# Autodesk Inventor assembly: Carriage_Assembly
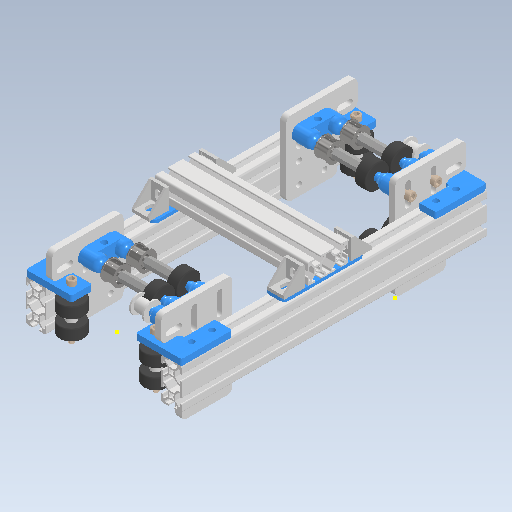
[picture p0: Inventor's stored thumbnail of the model, 512x512]
Saved by Autodesk Inventor 2021 (Build 250183000, 183)
## iProperties
Created: 2021-09-08
Part Number: Carriage_Assembly
Document SubType Name: Assembly
Designer: Jorian Brusind
Author: Jorian Brusind
## Documents named in this file (13)
- C:\Users\Jorian Brusind\Documents\GitHub\HyperRail\Inventor Files\Carriage_Assembly.iam
- C:\Users\Jorian Brusind\Documents\GitHub\PersonalProjects\HyperRail\Inventor Files\8020_Sets\IPT_20_Series\IPT_20_Series\20-2040_150mm.ipt
- C:\Users\Jorian Brusind\Documents\GitHub\HyperRail\Inventor Files\X_CarriageR_V2_0.iam
- C:\Users\Jorian Brusind\Documents\GitHub\HyperRail\Inventor Files\X_Carriage_V2_0.iam
- C:\Users\Jorian Brusind\Documents\GitHub\HyperRail\Inventor Files\8020_Sets\IPT_20_Series\Extra_20_Series\8020_14056m\14056_m.ipt
- C:\Users\Jorian Brusind\Documents\GitHub\HyperRail\Inventor Files\Buffer.iam
- C:\Users\Jorian Brusind\Documents\GitHub\HyperRail\Inventor Files\Metric Spacer_Standoffs\hex spacer standoff nut M5 L30.ipt
- C:\Users\Jorian Brusind\Documents\GitHub\HyperRail\Inventor Files\Carriage_Horizontal_Spacer.ipt
- C:\Users\Jorian Brusind\Documents\GitHub\PersonalProjects\HyperRail\Inventor Files\8020_Sets\IPT_20_Series\IPT_20_Series\20-2040_400mm.ipt
- C:\Users\Jorian Brusind\Documents\GitHub\HyperRail\Inventor Files\X_CarriageL_V2_1_Short.iam
- C:\Users\Jorian Brusind\Documents\GitHub\HyperRail\Inventor Files\X_CarriageR_V2_1_Short.iam
- C:\Users\Jorian Brusind\Documents\GitHub\HyperRail\Inventor Files\Buffer_L.iam
- C:\Users\Jorian Brusind\Documents\GitHub\HyperRail\Inventor Files\Metric bolt\Bolt M5 45mm.ipt
## Components (25 placed, 12 different names)
1. 20-2040_150mm:1 — Mate:20, Mate:21, Mate:22, Mate:23, Mate:80, Flush:33
2. X_CarriageR_V2_0:1 [sub-assembly] — Mate:96, Flush:56, Flush:61, Flush:63, Flush:65, Flush:67, Mate:122, Mate:124, Mate:126, Mate:127, Mate:134, Mate:143, Mate:144, Mate:145, Mate:146
3. 14056_m:1 — Mate:21, Flush:26, Flush:38, Mate:122
4. 14056_m:2 — Mate:20, Flush:25, Flush:26, Mate:70, Flush:37, Flush:39
5. 14056_m:3 — Mate:22, Flush:13
6. 14056_m:4 — Mate:23, Flush:13, Flush:28, Mate:72
7. Buffer:2 [sub-assembly] — Mate:86, Flush:47, Flush:55
8. Buffer:3 [sub-assembly] — Flush:42, Mate:87, Flush:43
9. Carriage_Horizontal_Spacer:1 — Flush:28, Mate:72, Mate:79, Mate:80
10. Carriage_Horizontal_Spacer:2 — Flush:25, Mate:70, Mate:84, Flush:37, Flush:38
11. 20-2040_400mm:1 — Flush:30, Mate:75, Mate:76, Mate:79, Flush:33, Flush:36, Mate:86, Flush:47, Flush:55, Mate:111, Mate:112, Flush:59, Flush:60, Flush:68, Mate:140, Flush:71, Flush:72
12. 20-2040_400mm:2 — Flush:30, Flush:36, Mate:84, Flush:39, Flush:42, Mate:87, Flush:43, Mate:96, Mate:107, Mate:139, Flush:69, Flush:70
13. X_Carriage_V2_0:2 [sub-assembly] — Mate:107, Flush:63, Flush:64, Flush:65, Flush:67, Mate:130, Mate:131, Mate:138
14. X_CarriageL_V2_1_Short:1 [sub-assembly] — Mate:112, Flush:57, Flush:60, Flush:61, Flush:66, Mate:132, Mate:133, Mate:141, Mate:142, Mate:147, Mate:148
15. X_CarriageR_V2_1_Short:1 [sub-assembly] — Mate:111, Flush:56, Flush:57, Flush:59, Flush:64, Flush:66, Flush:68, Mate:135, Mate:136, Mate:137
16. hex spacer standoff nut M5 L30:1 — Mate:124, Mate:126, Mate:133
17. hex spacer standoff nut M5 L30:2 — Mate:130, Mate:135
18. hex spacer standoff nut M5 L30:3 — Mate:127, Mate:132, Mate:134
19. hex spacer standoff nut M5 L30:4 — Mate:131, Mate:136, Mate:137, Mate:138
20. Buffer_L:1 [sub-assembly] — Mate:139, Flush:69, Flush:70
21. Buffer_L:2 [sub-assembly] — Mate:140, Flush:71, Flush:72
22. Bolt M5 45mm:1 — Mate:142, Mate:148
23. Bolt M5 45mm:2 — Mate:141, Mate:147
24. Bolt M5 45mm:3 — Mate:143, Mate:145
25. Bolt M5 45mm:4 — Mate:144, Mate:146
## Relationships (69: Mate 40, Flush 29)
- Mate:20 (3 mm): 20-2040_150mm:1 ↔ 14056_m:2
- Mate:21 (3 mm): 20-2040_150mm:1 ↔ 14056_m:1
- Mate:22 (3 mm): 20-2040_150mm:1 ↔ 14056_m:3
- Mate:23 (3 mm): 20-2040_150mm:1 ↔ 14056_m:4
- Flush:13: 14056_m:3 ↔ 14056_m:4
- Flush:25: 14056_m:2 ↔ Carriage_Horizontal_Spacer:2
- Flush:26: 14056_m:1 ↔ 14056_m:2
- Mate:70: 14056_m:2 ↔ Carriage_Horizontal_Spacer:2
- Flush:28 (3 mm): 14056_m:4 ↔ Carriage_Horizontal_Spacer:1
- Mate:72: 14056_m:4 ↔ Carriage_Horizontal_Spacer:1
- Flush:30: 20-2040_400mm:1 ↔ 20-2040_400mm:2
- Mate:75: 20-2040_400mm:1
- Mate:76: 20-2040_400mm:1
- Mate:79: Carriage_Horizontal_Spacer:1 ↔ 20-2040_400mm:1
- Mate:80: 20-2040_150mm:1 ↔ Carriage_Horizontal_Spacer:1
- Flush:33: 20-2040_150mm:1 ↔ 20-2040_400mm:1
- Flush:36: 20-2040_400mm:1 ↔ 20-2040_400mm:2
- Mate:84: Carriage_Horizontal_Spacer:2 ↔ 20-2040_400mm:2
- Flush:37: 14056_m:2 ↔ Carriage_Horizontal_Spacer:2
- Flush:38: 14056_m:1 ↔ Carriage_Horizontal_Spacer:2
- Flush:39: 14056_m:2 ↔ 20-2040_400mm:2
- Mate:86: Buffer:2 ↔ 20-2040_400mm:1
- Flush:42: Buffer:3 ↔ 20-2040_400mm:2
- Mate:87: Buffer:3 ↔ 20-2040_400mm:2
- Flush:43: Buffer:3 ↔ 20-2040_400mm:2
- Flush:47: Buffer:2 ↔ 20-2040_400mm:1
- Mate:96: X_CarriageR_V2_0:1 ↔ 20-2040_400mm:2
- Flush:55: Buffer:2 ↔ 20-2040_400mm:1
- Mate:107: 20-2040_400mm:2 ↔ X_Carriage_V2_0:2
- Mate:111: 20-2040_400mm:1 ↔ X_CarriageR_V2_1_Short:1
- Flush:56: X_CarriageR_V2_0:1 ↔ X_CarriageR_V2_1_Short:1
- Mate:112: 20-2040_400mm:1 ↔ X_CarriageL_V2_1_Short:1
- Flush:57: X_CarriageL_V2_1_Short:1 ↔ X_CarriageR_V2_1_Short:1
- Flush:59: 20-2040_400mm:1 ↔ X_CarriageR_V2_1_Short:1
- Flush:60: 20-2040_400mm:1 ↔ X_CarriageL_V2_1_Short:1
- Flush:61: X_CarriageR_V2_0:1 ↔ X_CarriageL_V2_1_Short:1
- Flush:63: X_CarriageR_V2_0:1 ↔ X_Carriage_V2_0:2
- Flush:64: X_Carriage_V2_0:2 ↔ X_CarriageR_V2_1_Short:1
- Flush:65: X_CarriageR_V2_0:1 ↔ X_Carriage_V2_0:2
- Flush:66: X_CarriageL_V2_1_Short:1 ↔ X_CarriageR_V2_1_Short:1
- Flush:67: X_CarriageR_V2_0:1 ↔ X_Carriage_V2_0:2
- Flush:68: 20-2040_400mm:1 ↔ X_CarriageR_V2_1_Short:1
- Mate:122 (40 mm): X_CarriageR_V2_0:1 ↔ 14056_m:1
- Mate:124: X_CarriageR_V2_0:1 ↔ hex spacer standoff nut M5 L30:1
- Mate:126: X_CarriageR_V2_0:1 ↔ hex spacer standoff nut M5 L30:1
- Mate:127: X_CarriageR_V2_0:1 ↔ hex spacer standoff nut M5 L30:3
- Mate:130: X_Carriage_V2_0:2 ↔ hex spacer standoff nut M5 L30:2
- Mate:131: X_Carriage_V2_0:2 ↔ hex spacer standoff nut M5 L30:4
- Mate:132: X_CarriageL_V2_1_Short:1 ↔ hex spacer standoff nut M5 L30:3
- Mate:133: X_CarriageL_V2_1_Short:1 ↔ hex spacer standoff nut M5 L30:1
- Mate:134: X_CarriageR_V2_0:1 ↔ hex spacer standoff nut M5 L30:3
- Mate:135: X_CarriageR_V2_1_Short:1 ↔ hex spacer standoff nut M5 L30:2
- Mate:136: X_CarriageR_V2_1_Short:1 ↔ hex spacer standoff nut M5 L30:4
- Mate:137: X_CarriageR_V2_1_Short:1 ↔ hex spacer standoff nut M5 L30:4
- Mate:138: X_Carriage_V2_0:2 ↔ hex spacer standoff nut M5 L30:4
- Mate:139: 20-2040_400mm:2 ↔ Buffer_L:1
- Flush:69: 20-2040_400mm:2 ↔ Buffer_L:1
- Flush:70: 20-2040_400mm:2 ↔ Buffer_L:1
- Mate:140: 20-2040_400mm:1 ↔ Buffer_L:2
- Flush:71: 20-2040_400mm:1 ↔ Buffer_L:2
- Flush:72: 20-2040_400mm:1 ↔ Buffer_L:2
- Mate:141: X_CarriageL_V2_1_Short:1 ↔ Bolt M5 45mm:2
- Mate:142: X_CarriageL_V2_1_Short:1 ↔ Bolt M5 45mm:1
- Mate:143: X_CarriageR_V2_0:1 ↔ Bolt M5 45mm:3
- Mate:144: X_CarriageR_V2_0:1 ↔ Bolt M5 45mm:4
- Mate:145: X_CarriageR_V2_0:1 ↔ Bolt M5 45mm:3
- Mate:146: X_CarriageR_V2_0:1 ↔ Bolt M5 45mm:4
- Mate:147: X_CarriageL_V2_1_Short:1 ↔ Bolt M5 45mm:2
- Mate:148: X_CarriageL_V2_1_Short:1 ↔ Bolt M5 45mm:1
